# Autodesk Inventor assembly: motor holder
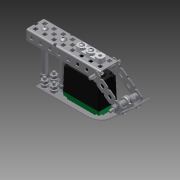
[picture p0: Inventor's stored thumbnail of the model, 180x180]
Saved by Autodesk Inventor 2014 SP1 (Build 180222100, 222)
## iProperties
Created: 2013-10-24
Part Number: motor holder
Document SubType Name: Assembly
Designer: RyanHughes
Author: RyanHughes
## Documents named in this file (16)
- C:\Users\Ryan\Desktop\sw\toss up 2ed A bot\intake\motor holder.iam
- C:\Users\Ryan\Desktop\sw\lib\Aperture VEX CAD Library\Metal\C Channel\2 x 8.ipt
- C:\Users\Ryan\Desktop\sw\lib\Aperture VEX CAD Library\Hardware\8-32\8-32 Nylock.ipt
- C:\Users\Ryan\Desktop\sw\lib\Aperture VEX CAD Library\Standoffs\BEAM-2000.ipt
- C:\Users\Ryan\Desktop\sw\lib\Aperture VEX CAD Library\Hardware\8-32\8-32_.500.ipt
- C:\Users\Ryan\Desktop\sw\lib\Aperture VEX CAD Library\Hardware\8-32\8-32_.375.ipt
- C:\Users\Ryan\Desktop\sw\lib\Super Sonic Sparks VEX CAD Library\Motors & Sensors\2-Wire Motor 393-Without Wire.iam
- C:\Users\Ryan\Desktop\sw\lib\Aperture VEX CAD Library\Bearing Blocks\Bearing Block.ipt
- C:\Users\Ryan\Desktop\sw\lib\Aperture VEX CAD Library\Hardware\6-32\6-32_.500.ipt
- C:\Users\Ryan\Desktop\sw\lib\Aperture VEX CAD Library\Metal\Custom 1 bar\4 holes.ipt
- C:\Users\Ryan\Desktop\sw\lib\Aperture VEX CAD Library\Bearing Blocks\Pillow Block.ipt
- C:\Users\Ryan\Desktop\sw\toss up 2ed A bot\intake\ski poly.ipt
- C:\Users\Ryan\Desktop\sw\lib\Aperture VEX CAD Library\Spacers\thin\SPACER-0320-0375.ipt
- C:\Users\Ryan\Desktop\sw\lib\Aperture VEX CAD Library\Hardware\8-32\8-32_1.500.ipt
- C:\Users\Ryan\Desktop\sw\lib\Aperture VEX CAD Library\Spacers\thin\SPACER-0320-0125.ipt
- C:\Users\Ryan\Desktop\sw\lib\Aperture VEX CAD Library\Hardware\6-32\thinner locknut.iam
## Components (41 placed, 15 different names)
1. 2 x 8:1 — Mate:1, Mate:2, Mate:3, Mate:4, Mate:5, Mate:6, Mate:9, Mate:10, Mate:20, Mate:21, Mate:23, Mate:24, Mate:25, Mate:26, Mate:27, Mate:34, Mate:35, Mate:36, Mate:37, Mate:46, Mate:47, Mate:48, Mate:49, Mate:52, Mate:53, Mate:54
2. 8-32 Nylock:1 — Mate:1, Mate:2, Mate:3, Mate:8, Mate:22
3. 8-32 Nylock:2 — Mate:4, Mate:5, Mate:6, Mate:7, Mate:19
4. BEAM-2000:1 — Mate:7, Mate:9, Mate:13, Mate:14
5. BEAM-2000:2 — Mate:8, Mate:10, Mate:11, Mate:12
6. 8-32 Nylock:3 — Mate:11, Mate:12, Mate:17, Mate:18
7. 8-32 Nylock:4 — Mate:13, Mate:14, Mate:15, Mate:16
8. 8-32_.500:1 — Mate:15, Mate:16, Flush:2
9. 8-32_.500:2 — Mate:17, Mate:18
10. 8-32_.375:1 — Mate:19, Mate:20
11. 8-32_.375:2 — Mate:21, Mate:22
12. 2-Wire Motor 393-Without Wire:1 [sub-assembly] — Mate:23, Mate:24, Mate:25, Mate:26, Mate:28, Mate:29
13. Bearing Block:1 — Mate:27, Mate:28, Mate:29, Mate:30, Mate:31, Mate:33, Mate:32
14. 6-32_.500:1 — Mate:31, Mate:32
15. 6-32_.500:2 — Mate:30, Mate:33
16. 4 holes:1 — Mate:34, Mate:38, Mate:39, Flush:1, Mate:50, Mate:51, Mate:60, Mate:64
17. 8-32_.375:3 — Mate:35, Mate:36, Mate:37, Mate:38, Mate:39
18. 4 holes:2 — Mate:47, Flush:1, Mate:62, Mate:65
19. 8-32_.375:4 — Mate:46, Mate:48, Mate:49
20. Pillow Block:1 — Mate:50, Mate:51, Mate:55, Mate:57, Mate:59, Mate:71, Mate:74
21. ski poly:1 — Mate:52, Mate:53, Mate:54, Flush:2, Mate:55, Angle:2, Mate:58, Mate:67, Mate:68, Mate:69, Mate:70, Mate:78, Mate:81, Mate:89
22. SPACER-0320-0375:1 — Mate:59, Mate:60, Mate:61, Mate:63
23. SPACER-0320-0375:2 — Mate:61, Mate:62
24. 8-32_1.500:1 — Mate:63, Mate:64, Mate:66
25. 8-32 Nylock:7 — Mate:65, Mate:66
26. 8-32_.375:5 — Mate:67, Mate:68, Mate:72
27. 8-32_.375:6 — Mate:69, Mate:70, Mate:73
28. 8-32 Nylock:8 — Mate:73, Mate:74
29. 8-32 Nylock:9 — Mate:71, Mate:72
30. SPACER-0320-0125:2 — Mate:85, Mate:89, Mate:91
31. thinner locknut:1 [sub-assembly] — Mate:91, Mate:92
32. 6-32_.500:6 — Mate:78, Mate:81, Mate:85, Mate:92
33. SPACER-0320-0125:3
34. thinner locknut:2 [sub-assembly]
35. 6-32_.500:7
36. SPACER-0320-0125:4
37. thinner locknut:3 [sub-assembly]
38. 6-32_.500:8
39. SPACER-0320-0125:5
40. thinner locknut:4 [sub-assembly]
41. 6-32_.500:9
## Component patterns: (4 elements, first: SPACER-0320-0125:2 + thinner locknut:1 + 6-32_.500:6)
## Relationships (78: Mate 75, Flush 2, Angle 1)
- Mate:1: 2 x 8:1 ↔ 8-32 Nylock:1
- Mate:2 (2.3114 mm): 2 x 8:1 ↔ 8-32 Nylock:1
- Mate:3 (2.3114 mm): 2 x 8:1 ↔ 8-32 Nylock:1
- Mate:4 (2.3114 mm): 2 x 8:1 ↔ 8-32 Nylock:2
- Mate:5 (2.3114 mm): 2 x 8:1 ↔ 8-32 Nylock:2
- Mate:6: 2 x 8:1 ↔ 8-32 Nylock:2
- Mate:7: 8-32 Nylock:2 ↔ BEAM-2000:1
- Mate:8: 8-32 Nylock:1 ↔ BEAM-2000:2
- Mate:9: 2 x 8:1 ↔ BEAM-2000:1
- Mate:10: 2 x 8:1 ↔ BEAM-2000:2
- Mate:11: BEAM-2000:2 ↔ 8-32 Nylock:3
- Mate:12: BEAM-2000:2 ↔ 8-32 Nylock:3
- Mate:13: BEAM-2000:1 ↔ 8-32 Nylock:4
- Mate:14: BEAM-2000:1 ↔ 8-32 Nylock:4
- Mate:15 (1.5875 mm): 8-32 Nylock:4 ↔ 8-32_.500:1
- Mate:16: 8-32 Nylock:4 ↔ 8-32_.500:1
- Mate:17: 8-32 Nylock:3 ↔ 8-32_.500:2
- Mate:18 (1.5875 mm): 8-32 Nylock:3 ↔ 8-32_.500:2
- Mate:19: 8-32 Nylock:2 ↔ 8-32_.375:1
- Mate:20: 2 x 8:1 ↔ 8-32_.375:1
- Mate:21: 2 x 8:1 ↔ 8-32_.375:2
- Mate:22: 8-32 Nylock:1 ↔ 8-32_.375:2
- Mate:23: 2 x 8:1 ↔ 2-Wire Motor 393-Without Wire:1
- Mate:24 (2.3114 mm): 2 x 8:1 ↔ 2-Wire Motor 393-Without Wire:1
- Mate:25 (2.3114 mm): 2 x 8:1 ↔ 2-Wire Motor 393-Without Wire:1
- Mate:26 (2.3114 mm): 2 x 8:1 ↔ 2-Wire Motor 393-Without Wire:1
- Mate:27: 2 x 8:1 ↔ Bearing Block:1
- Mate:28: 2-Wire Motor 393-Without Wire:1 ↔ Bearing Block:1
- Mate:29: 2-Wire Motor 393-Without Wire:1 ↔ Bearing Block:1
- Mate:30: Bearing Block:1 ↔ 6-32_.500:2
- Mate:31: Bearing Block:1 ↔ 6-32_.500:1
- Mate:32: Bearing Block:1 ↔ 6-32_.500:1
- Mate:33: Bearing Block:1 ↔ 6-32_.500:2
- Mate:34: 2 x 8:1 ↔ 4 holes:1
- Mate:35: 2 x 8:1 ↔ 8-32_.375:3
- Mate:36 (2.3114 mm): 2 x 8:1 ↔ 8-32_.375:3
- Mate:37 (2.3114 mm): 2 x 8:1 ↔ 8-32_.375:3
- Mate:38 (2.3114 mm): 4 holes:1 ↔ 8-32_.375:3
- Mate:39 (2.3114 mm): 4 holes:1 ↔ 8-32_.375:3
- [Mate] (2.3114 mm): 4 holes:2 ↔ 8-32_.375:4
- [Mate] (2.3114 mm): 4 holes:2 ↔ 8-32_.375:4
- Mate:46: 2 x 8:1 ↔ 8-32_.375:4
- Mate:47: 2 x 8:1 ↔ 4 holes:2
- Mate:48 (2.3114 mm): 2 x 8:1 ↔ 8-32_.375:4
- Mate:49 (2.3114 mm): 2 x 8:1 ↔ 8-32_.375:4
- Flush:1: 4 holes:1 ↔ 4 holes:2
- Mate:50 (2.3114 mm): 4 holes:1 ↔ Pillow Block:1
- Mate:51 (2.3114 mm): 4 holes:1 ↔ Pillow Block:1
- Mate:52 (2.3114 mm): 2 x 8:1 ↔ ski poly:1
- Mate:53 (2.3114 mm): 2 x 8:1 ↔ ski poly:1
- Mate:54 (2.3114 mm): 2 x 8:1 ↔ ski poly:1
- Flush:2 (3.175 mm): 8-32_.500:1 ↔ ski poly:1
- Mate:55: Pillow Block:1 ↔ ski poly:1
- Mate:57: Pillow Block:1
- Angle:2 (0 deg): ski poly:1
- Mate:58 (-4.9784 mm): ski poly:1
- Mate:59: Pillow Block:1 ↔ SPACER-0320-0375:1
- Mate:60: 4 holes:1 ↔ SPACER-0320-0375:1
- Mate:61: SPACER-0320-0375:1 ↔ SPACER-0320-0375:2
- Mate:62: 4 holes:2 ↔ SPACER-0320-0375:2
- Mate:63: SPACER-0320-0375:1 ↔ 8-32_1.500:1
- Mate:64: 4 holes:1 ↔ 8-32_1.500:1
- Mate:65: 4 holes:2 ↔ 8-32 Nylock:7
- Mate:66: 8-32_1.500:1 ↔ 8-32 Nylock:7
- Mate:67: ski poly:1 ↔ 8-32_.375:5
- Mate:68: ski poly:1 ↔ 8-32_.375:5
- Mate:69: ski poly:1 ↔ 8-32_.375:6
- Mate:70: ski poly:1 ↔ 8-32_.375:6
- Mate:71: Pillow Block:1 ↔ 8-32 Nylock:9
- Mate:72: 8-32_.375:5 ↔ 8-32 Nylock:9
- Mate:73: 8-32_.375:6 ↔ 8-32 Nylock:8
- Mate:74: Pillow Block:1 ↔ 8-32 Nylock:8
- Mate:78: ski poly:1 ↔ 6-32_.500:6
- Mate:81: ski poly:1 ↔ 6-32_.500:6
- Mate:85: SPACER-0320-0125:2 ↔ 6-32_.500:6
- Mate:89: ski poly:1 ↔ SPACER-0320-0125:2
- Mate:91 (1.5875 mm): SPACER-0320-0125:2 ↔ thinner locknut:1
- Mate:92: thinner locknut:1 ↔ 6-32_.500:6
## Named parameters: q = 2.3114 mm, d47_d43 = 2.3114 mm, d48_d44 = 2.3114 mm, d51_q = 2.3114 mm
